# Autodesk Inventor assembly: 3D_Scanner_Prototyp
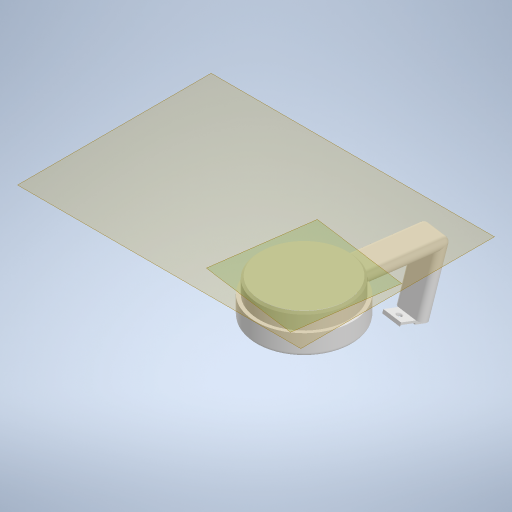
[picture p0: Inventor's stored thumbnail of the model, 512x512]
Saved by Autodesk Inventor 2023 (Build 270158000, 158)
## iProperties
Created: 2022-06-11
Part Number: 3D_Scanner_Prototyp
Document SubType Name: Assembly
Designer: Habib
Author: Habib
## Documents named in this file (4)
- C:\Users\Habib\OneDrive\Bureau\3D-Scanner\Konstruktion\3D_Scanner_Prototyp.iam
- C:\Users\Habib\OneDrive\Bureau\3D-Scanner\Konstruktion\Gehaeuse_prototyp.ipt
- C:\Users\Habib\OneDrive\Bureau\3D-Scanner\Konstruktion\Kamerahalter_prototyp.ipt
- C:\Users\Habib\OneDrive\Bureau\3D-Scanner\Konstruktion\Drehplatform_prototyp.ipt
## Components (3 placed, 3 different names)
1. Gehaeuse_prototyp:1 — Mate:1, Flush:1, Mate:2, Insert:1, Mate:3
2. Kamerahalter_prototyp:1 — Mate:1, Flush:1, Mate:2
3. Drehplatform_prototyp:1 — Insert:1
## Relationships (5: Mate 3, Flush 1, Insert 1)
- Mate:1: Gehaeuse_prototyp:1 ↔ Kamerahalter_prototyp:1
- Flush:1: Gehaeuse_prototyp:1 ↔ Kamerahalter_prototyp:1
- Mate:2 (15 mm): Gehaeuse_prototyp:1 ↔ Kamerahalter_prototyp:1
- Insert:1: Gehaeuse_prototyp:1 ↔ Drehplatform_prototyp:1
- Mate:3: Gehaeuse_prototyp:1
